# Autodesk Inventor assembly: silnik_full_assembly
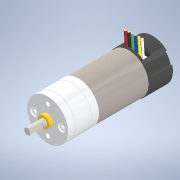
[picture p0: Inventor's stored thumbnail of the model, 180x180]
Saved by Autodesk Inventor 2020 (Build 240168000, 168)
## iProperties
Created: 2020-05-04
Part Number: silnik_full_assembly
Document SubType Name: Assembly
Designer: Hesekiel
Author: Hesekiel
## Documents named in this file (3)
- C:\Users\Hesekiel\Documents\Inventor\Uchwyt Aktywny Teleskopu\silnik_full_assembly.iam
- C:\Users\Hesekiel\Documents\Inventor\Uchwyt Aktywny Teleskopu\wal_silnika.ipt
- C:\Users\Hesekiel\Documents\Inventor\Uchwyt Aktywny Teleskopu\Silnik.ipt
## Components (2 placed, 2 different names)
1. wal_silnika:1 — Rotational:1
2. Silnik:1 — Rotational:1
## Relationships (1: RevoluteJoint 1)
- Rotational:1 [RevoluteJoint]: wal_silnika:1 ↔ Silnik:1
